# Autodesk Inventor assembly: PossibleClaw1
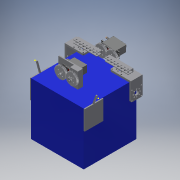
[picture p0: Inventor's stored thumbnail of the model, 180x180]
Saved by Autodesk Inventor 2017 (Build 210142000, 142)
## iProperties
Created: 2017-09-20
Part Number: PossibleClaw1
Document SubType Name: Assembly
Designer: User
Author: User
## Documents named in this file (9)
- C:\Robotics\CAD\2017-18_CAD\PossibleClaw1.iam
- C:\Robotics\CAD\2017-18_CAD\Glyph6x6x6.ipt
- C:\Robotics\CAD\COTSParts\Actobotics\585 parts\585494.ipt
- C:\Robotics\CAD\COTSParts\Actobotics\585 parts\585382.ipt
- C:\Robotics\CAD\COTSParts\Tetrix\Tetrix Gear 40T.ipt
- C:\Robotics\CAD\COTSParts\Tetrix\Tetrix servo 180.ipt
- C:\Robotics\CAD\2017-18_CAD\ClawPaddle.ipt
- C:\Robotics\CAD\2017-18_CAD\ClawServoHolder.ipt
- C:\Robotics\CAD\COTSParts\Vex\91259A574_ALLOY STEEL SHOULDER SCREW.ipt
## Components (15 placed, 8 different names)
1. Glyph6x6x6:1 — Mate:1, Flush:4, Mate:2, Flush:5, Flush:6, Mate:3, Flush:7, Flush:8, Mate:4
2. 585494:1 — Flush:3, Insert:7, Flush:4, Mate:2
3. 585494:2 — Flush:3, Insert:1, Insert:2, Mate:1
4. 585382:2 — Insert:5, Insert:7
5. 585382:3 — Insert:1, Insert:2, Insert:6
6. Tetrix Gear 40T:1 — Insert:6, Tangent:1, Insert:8, Insert:9
7. Tetrix Gear 40T:2 — Insert:5, Tangent:1
8. Tetrix servo 180:1 — Insert:8, Insert:9
9. ClawPaddle:1 — Flush:5, Flush:6, Mate:3, Mate:5, Flush:10
10. ClawPaddle:3 — Flush:7, Flush:8, Mate:4, Flush:9
11. ClawServoHolder:1 — Flush:9, Insert:14, Insert:15, Mate:5, Flush:10, Insert:18
12. Tetrix servo 180:2 — Insert:14, Insert:15, Mate:6, Insert:16, Insert:17
13. Tetrix Gear 40T:3 — Tangent:2, Tangent:3, Flush:11, Insert:18, Insert:19
14. Tetrix Gear 40T:4 — Tangent:2, Tangent:3, Flush:11, Mate:6, Insert:16, Insert:17
15. 91259A574_ALLOY STEEL SHOULDER SCREW:1 — Insert:19
## Relationships (31: Insert 13, Flush 9, Mate 6, Tangent 3)
- Flush:3: 585494:1 ↔ 585494:2
- Insert:1: 585494:2 ↔ 585382:3
- Insert:2: 585494:2 ↔ 585382:3
- Insert:5: 585382:2 ↔ Tetrix Gear 40T:2
- Insert:6: 585382:3 ↔ Tetrix Gear 40T:1
- Tangent:1: Tetrix Gear 40T:1 ↔ Tetrix Gear 40T:2
- Insert:7: 585494:1 ↔ 585382:2
- Mate:1 (12.7 mm): Glyph6x6x6:1 ↔ 585494:2
- Flush:4: Glyph6x6x6:1 ↔ 585494:1
- Mate:2 (12.7 mm): Glyph6x6x6:1 ↔ 585494:1
- Insert:8: Tetrix Gear 40T:1 ↔ Tetrix servo 180:1
- Insert:9: Tetrix Gear 40T:1 ↔ Tetrix servo 180:1
- Flush:5: Glyph6x6x6:1 ↔ ClawPaddle:1
- Flush:6: Glyph6x6x6:1 ↔ ClawPaddle:1
- Mate:3: Glyph6x6x6:1 ↔ ClawPaddle:1
- Flush:7: Glyph6x6x6:1 ↔ ClawPaddle:3
- Flush:8: Glyph6x6x6:1 ↔ ClawPaddle:3
- Mate:4: Glyph6x6x6:1 ↔ ClawPaddle:3
- Flush:9 (65.8622 mm): ClawPaddle:3 ↔ ClawServoHolder:1
- Insert:14: ClawServoHolder:1 ↔ Tetrix servo 180:2
- Insert:15: ClawServoHolder:1 ↔ Tetrix servo 180:2
- Mate:5: ClawPaddle:1 ↔ ClawServoHolder:1
- Flush:10: ClawPaddle:1 ↔ ClawServoHolder:1
- Tangent:2: Tetrix Gear 40T:3 ↔ Tetrix Gear 40T:4
- Tangent:3: Tetrix Gear 40T:3 ↔ Tetrix Gear 40T:4
- Flush:11: Tetrix Gear 40T:3 ↔ Tetrix Gear 40T:4
- Mate:6 (6.35 mm): Tetrix servo 180:2 ↔ Tetrix Gear 40T:4
- Insert:16: Tetrix servo 180:2 ↔ Tetrix Gear 40T:4
- Insert:17: Tetrix servo 180:2 ↔ Tetrix Gear 40T:4
- Insert:18: ClawServoHolder:1 ↔ Tetrix Gear 40T:3
- Insert:19: Tetrix Gear 40T:3 ↔ 91259A574_ALLOY STEEL SHOULDER SCREW:1
